# Autodesk Inventor assembly: forklift_1_0
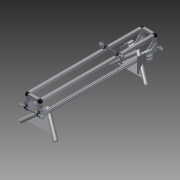
[picture p0: Inventor's stored thumbnail of the model, 180x180]
Saved by Autodesk Inventor 2011 (Build 150239000, 239)
## iProperties
Created: 2013-01-16
Part Number: forklift_1_0
Document SubType Name: Assembly
Designer: 917788
Author: 917788
## Documents named in this file (17)
- F:\Users\Christopher\Documents\GitHub\2013CAD\2013 robot\forklift\frame parts\forklift_1_0.iam
- F:\Users\Christopher\Documents\GitHub\2013CAD\2013 robot\forklift\frame parts\1tube_6.ipt
- F:\Users\Christopher\Documents\GitHub\2013CAD\2013 robot\forklift\frame parts\1tube_9.ipt
- F:\Users\Christopher\Documents\GitHub\2013CAD\2013 robot\forklift\frame parts\1tube_40.ipt
- F:\Users\Christopher\Documents\GitHub\2013CAD\2013 robot\forklift\frame parts\8020_40.ipt
- F:\Users\Christopher\Documents\GitHub\2013CAD\2013 robot\forklift\frame parts\8020_gussetplate.ipt
- F:\Users\Christopher\Documents\GitHub\2013CAD\2013 robot\forklift\Misc parts\3-way corner.ipt
- F:\Users\Christopher\Documents\GitHub\2013CAD\2013 robot\forklift\Misc parts\1.5_bolt_.25_20.ipt
- F:\Users\Christopher\Documents\GitHub\2013CAD\2013 robot\forklift\Misc parts\2_bolt_.25_20.ipt
- F:\Users\Christopher\Documents\GitHub\2013CAD\2013 robot\forklift\Misc parts\nut_.25_20.ipt
- F:\Users\Christopher\Documents\GitHub\2013CAD\2013 robot\forklift\frame parts\hook_right.iam
- F:\Users\Christopher\Documents\GitHub\2013CAD\2013 robot\forklift\frame parts\hook_left.iam
- F:\Users\Christopher\Documents\GitHub\2013CAD\2013 robot\forklift\Misc parts\.5inch_side_bearing.ipt
- F:\Users\Christopher\Documents\GitHub\2013CAD\2013 robot\forklift\frame parts\0.5unkeyedaxle_11.ipt
- F:\Users\Christopher\Documents\GitHub\2013CAD\2013 robot\forklift\Misc parts\.5_inch_axle_bushing.ipt
- F:\Users\Christopher\Documents\GitHub\2013CAD\2013 robot\forklift\frame parts\1.5inch_sprocket.ipt
- F:\Users\Christopher\Documents\GitHub\2013CAD\2013 robot\forklift\frame parts\corner_prop.ipt
## Components (137 placed, 16 different names)
1. 1tube_9:1 — Mate:9, Mate:10, Flush:8, Mate:11, Mate:12, Flush:9, Insert:3, Insert:4, Insert:44, Insert:51
2. 1tube_40:1 — Mate:7, Flush:7, Mate:8, Mate:20, Mate:21, Flush:18, Insert:2, Insert:12, Insert:43, Insert:136, Insert:137, Insert:144, Insert:145
3. 8020_40:1 — Flush:22, Flush:24, Mate:42, Flush:28, Mate:49, Flush:38, Flush:39, Mate:64, Mate:65
4. 8020_gussetplate:1 — Mate:50, Flush:40, Flush:41, Insert:84, Insert:85, Insert:86, Insert:87, Insert:88
5. 1tube_40:2 — Mate:13, Mate:14, Flush:10, Mate:22, Mate:23, Mate:24, Insert:6, Insert:8, Insert:52, Insert:58, Insert:138, Insert:139, Insert:146, Insert:147
6. 1tube_9:2 — Mate:25, Mate:26, Mate:27, Insert:9, Insert:10, Insert:67, Insert:71
7. 1tube_6:2 — Mate:1, Flush:4, Flush:5, Mate:46, Flush:36, Mate:48, Flush:37, Insert:1, Insert:42, Insert:77, Insert:104
8. 8020_40:2 — Mate:1, Flush:3, Flush:6, Flush:20, Flush:34, Mate:47, Flush:35, Flush:37, Mate:62, Mate:63
9. 8020_gussetplate:2 — Flush:24, Mate:43, Flush:31, Flush:32, Insert:53, Insert:54, Insert:55, Insert:56, Insert:57
10. 8020_gussetplate:3 — Mate:55, Flush:42, Flush:43, Insert:91, Insert:92, Insert:93, Insert:94, Insert:95
11. 8020_gussetplate:4 — Flush:5, Flush:6, Mate:46, Flush:36, Insert:89, Insert:90, Insert:96, Insert:97, Insert:98
12. 8020_gussetplate:5 — Flush:3, Flush:4, Mate:48, Insert:99, Insert:100, Insert:101, Insert:102, Insert:103
13. 8020_gussetplate:7 — Flush:22, Flush:29, Flush:30, Insert:32, Insert:33, Insert:34, Insert:35, Insert:36, Insert:158
14. 8020_gussetplate:8 — Mate:31, Flush:19, Flush:20, Insert:22, Insert:23, Insert:24, Insert:25, Insert:26
15. 8020_gussetplate:9 — Mate:37, Flush:25, Flush:26, Insert:60, Insert:61, Insert:62, Insert:63, Insert:64
16. 3-way corner:1 — Mate:11, Mate:12, Flush:9, Mate:13, Mate:14, Flush:10, Mate:52, Mate:53, Mate:54
17. 3-way corner:2 — Mate:7, Flush:7, Mate:8, Mate:9, Mate:10, Flush:8
18. 3-way corner:3 — Mate:20, Mate:21, Flush:18, Mate:25, Mate:28, Mate:29, Mate:30
19. 3-way corner:4 — Mate:22, Mate:23, Mate:24, Mate:26, Mate:27, Mate:44, Mate:51
20. 1tube_6:4 — Mate:28, Mate:29, Mate:30, Mate:31, Flush:19, Mate:37, Flush:25, Flush:26, Flush:34, Mate:47, Flush:35, Insert:11, Insert:68, Insert:111, Insert:112, Insert:119
21. 1tube_6:5 — Mate:42, Mate:43, Flush:28, Flush:29, Flush:30, Flush:31, Flush:32, Mate:44, Mate:51, Insert:7, Insert:59, Insert:113, Insert:114, Insert:120, Insert:158
22. 1tube_6:6 — Mate:49, Flush:38, Flush:39, Mate:50, Mate:52, Mate:53, Mate:54, Flush:40, Flush:41, Mate:55, Flush:42, Flush:43, Insert:5, Insert:50, Insert:73, Insert:105
23. 1.5_bolt_.25_20:1 — Insert:2
24. 1.5_bolt_.25_20:2 — Insert:1
25. 1.5_bolt_.25_20:3 — Insert:4
26. 1.5_bolt_.25_20:4 — Insert:3
27. 1.5_bolt_.25_20:5 — Insert:6
28. 1.5_bolt_.25_20:6 — Insert:11
29. 1.5_bolt_.25_20:7 — Insert:8
30. 1.5_bolt_.25_20:8 — Insert:9
31. 1.5_bolt_.25_20:9 — Insert:7
32. 1.5_bolt_.25_20:10 — Insert:10
33. 1.5_bolt_.25_20:13 — Insert:12
34. 1.5_bolt_.25_20:14 — Insert:5
35. 2_bolt_.25_20:8 — Insert:22
36. 2_bolt_.25_20:9 — Insert:23
37. 2_bolt_.25_20:10 — Insert:26
38. 2_bolt_.25_20:11 — Insert:24
39. 2_bolt_.25_20:12 — Insert:25
40. 2_bolt_.25_20:13 — Insert:35
41. 2_bolt_.25_20:14 — Insert:36
42. 2_bolt_.25_20:15 — Insert:34
43. 2_bolt_.25_20:16 — Insert:33
44. 2_bolt_.25_20:17 — Insert:32
45. nut_.25_20:4 — Insert:44
46. nut_.25_20:6 — Insert:50
47. nut_.25_20:7 — Insert:43
48. nut_.25_20:9 — Insert:52
49. nut_.25_20:10 — Insert:51
50. nut_.25_20:11 — Insert:53
51. nut_.25_20:17 — Insert:42
52. nut_.25_20:18 — Insert:63
53. nut_.25_20:19 — Insert:54
54. nut_.25_20:20 — Insert:61
55. nut_.25_20:21 — Insert:62
56. nut_.25_20:22 — Insert:57
57. nut_.25_20:23 — Insert:60
58. nut_.25_20:26 — Insert:59
59. nut_.25_20:27 — Insert:56
60. nut_.25_20:28 — Insert:64
61. nut_.25_20:30 — Insert:67
62. nut_.25_20:31 — Insert:55
63. nut_.25_20:33 — Insert:58
64. nut_.25_20:34 — Insert:71
65. nut_.25_20:35 — Insert:68
66. hook_right:1 [sub-assembly] — Flush:44, Flush:45, Mate:62, Mate:63
67. hook_left:1 [sub-assembly] — Flush:44, Mate:61, Mate:64, Mate:65
68. .5inch_side_bearing:3 — Insert:77, Insert:78, Insert:79, Insert:104, Insert:106, Insert:157
69. .5inch_side_bearing:4 — Insert:73, Insert:74, Insert:75, Insert:105, Insert:108
70. 1.5_bolt_.25_20:17 — Insert:78
71. 1.5_bolt_.25_20:18 — Insert:74
72. 1.5_bolt_.25_20:19 — Insert:75
73. 1.5_bolt_.25_20:20 — Insert:79
74. nut_.25_20:40 — Insert:95
75. 2_bolt_.25_20:18 — Insert:90
76. 2_bolt_.25_20:19 — Insert:84
77. 2_bolt_.25_20:20 — Insert:85
78. 2_bolt_.25_20:21 — Insert:86
79. 2_bolt_.25_20:22 — Insert:87
80. 2_bolt_.25_20:23 — Insert:96
81. 2_bolt_.25_20:24 — Insert:88
82. 2_bolt_.25_20:25 — Insert:89
83. 2_bolt_.25_20:28 — Insert:97
84. 2_bolt_.25_20:29 — Insert:98
85. nut_.25_20:41 — Insert:91
86. nut_.25_20:42 — Insert:92
87. nut_.25_20:43 — Insert:93
88. nut_.25_20:44 — Insert:101
89. nut_.25_20:45 — Insert:94
90. nut_.25_20:46 — Insert:102
91. nut_.25_20:47 — Insert:99
92. nut_.25_20:48 — Insert:103
93. nut_.25_20:49 — Insert:100
94. 0.5unkeyedaxle_11:1 — Insert:106, Insert:109, Insert:110
95. .5_inch_axle_bushing:1 — Insert:108
96. .5_inch_axle_bushing:2 — Insert:157
97. 1.5inch_sprocket:1 — Insert:109, Insert:122, Insert:124
98. 1.5inch_sprocket:2 — Insert:110, Insert:121, Insert:123
99. .5inch_side_bearing:5 — Insert:111, Insert:112, Insert:115, Insert:116, Insert:135
100. .5inch_side_bearing:6 — Insert:113, Insert:114, Insert:117, Insert:118, Insert:134
101. 1.5_bolt_.25_20:21 — Insert:115
102. 1.5_bolt_.25_20:22 — Insert:116
103. 1.5_bolt_.25_20:23 — Insert:117
104. 1.5_bolt_.25_20:24 — Insert:118
105. nut_.25_20:50 — Insert:119
106. nut_.25_20:51 — Insert:120
107. .5_inch_axle_bushing:3 — Insert:133
108. .5_inch_axle_bushing:4 — Insert:132
109. .5_inch_axle_bushing:5 — Insert:121
110. .5_inch_axle_bushing:6 — Insert:124
111. .5_inch_axle_bushing:7 — Insert:122
112. .5_inch_axle_bushing:8 — Insert:123
113. 1.5inch_sprocket:3 — Insert:128, Insert:131, Insert:132
114. 1.5inch_sprocket:4 — Insert:129, Insert:130, Insert:133
115. .5_inch_axle_bushing:9 — Insert:131
116. .5_inch_axle_bushing:10 — Insert:129, Insert:135
117. .5_inch_axle_bushing:11 — Insert:130
118. .5_inch_axle_bushing:12 — Insert:128, Insert:134
119. .5inch_side_bearing:7 — Insert:136, Insert:137, Insert:140, Insert:141, Insert:148
120. .5inch_side_bearing:8 — Insert:138, Insert:139, Insert:142, Insert:143
121. 1.5_bolt_.25_20:25 — Insert:140
122. 1.5_bolt_.25_20:26 — Insert:141
123. 1.5_bolt_.25_20:27 — Insert:142
124. 1.5_bolt_.25_20:28 — Insert:143
125. nut_.25_20:52 — Insert:146
126. nut_.25_20:53 — Insert:147
127. nut_.25_20:54 — Insert:145
128. nut_.25_20:55 — Insert:144
129. 0.5unkeyedaxle_11:2 — Insert:148, Insert:149, Insert:150, Insert:151
130. .5_inch_axle_bushing:13 — Insert:149
131. .5_inch_axle_bushing:14 — Insert:154
132. .5_inch_axle_bushing:15 — Insert:150, Insert:152
133. .5_inch_axle_bushing:17 — Insert:156
134. 1.5inch_sprocket:5 — Insert:151, Insert:156
135. 1.5inch_sprocket:6 — Insert:152, Insert:154
136. corner_prop:1 — Mate:61, Flush:45, Mate:66
137. corner_prop:2 — Mate:66
## Relationships (191: Insert 118, Mate 41, Flush 32)
- Mate:1: 1tube_6:2 ↔ 8020_40:2
- Flush:3: 8020_40:2 ↔ 8020_gussetplate:5
- Flush:4: 1tube_6:2 ↔ 8020_gussetplate:5
- Flush:5: 1tube_6:2 ↔ 8020_gussetplate:4
- Flush:6: 8020_40:2 ↔ 8020_gussetplate:4
- Mate:7: 1tube_40:1 ↔ 3-way corner:2
- Flush:7: 1tube_40:1 ↔ 3-way corner:2
- Mate:8: 1tube_40:1 ↔ 3-way corner:2
- Mate:9: 1tube_9:1 ↔ 3-way corner:2
- Mate:10: 1tube_9:1 ↔ 3-way corner:2
- Flush:8: 1tube_9:1 ↔ 3-way corner:2
- Mate:11: 1tube_9:1 ↔ 3-way corner:1
- Mate:12: 1tube_9:1 ↔ 3-way corner:1
- Flush:9: 1tube_9:1 ↔ 3-way corner:1
- Mate:13: 1tube_40:2 ↔ 3-way corner:1
- Mate:14: 1tube_40:2 ↔ 3-way corner:1
- Flush:10: 1tube_40:2 ↔ 3-way corner:1
- Mate:20: 1tube_40:1 ↔ 3-way corner:3
- Mate:21: 1tube_40:1 ↔ 3-way corner:3
- Flush:18: 1tube_40:1 ↔ 3-way corner:3
- Mate:22: 1tube_40:2 ↔ 3-way corner:4
- Mate:23: 1tube_40:2 ↔ 3-way corner:4
- Mate:24: 1tube_40:2 ↔ 3-way corner:4
- Mate:25: 1tube_9:2 ↔ 3-way corner:3
- Mate:26: 1tube_9:2 ↔ 3-way corner:4
- Mate:27: 1tube_9:2 ↔ 3-way corner:4
- Mate:28: 3-way corner:3 ↔ 1tube_6:4
- Mate:29: 3-way corner:3 ↔ 1tube_6:4
- Mate:30: 3-way corner:3 ↔ 1tube_6:4
- Mate:31: 8020_gussetplate:8 ↔ 1tube_6:4
- Flush:19: 8020_gussetplate:8 ↔ 1tube_6:4
- Flush:20: 8020_40:2 ↔ 8020_gussetplate:8
- Flush:22: 8020_40:1 ↔ 8020_gussetplate:7
- Flush:24: 8020_40:1 ↔ 8020_gussetplate:2
- Mate:37: 8020_gussetplate:9 ↔ 1tube_6:4
- Flush:25: 8020_gussetplate:9 ↔ 1tube_6:4
- Flush:26: 8020_gussetplate:9 ↔ 1tube_6:4
- Mate:42: 8020_40:1 ↔ 1tube_6:5
- Mate:43: 8020_gussetplate:2 ↔ 1tube_6:5
- Flush:28: 8020_40:1 ↔ 1tube_6:5
- Flush:29: 8020_gussetplate:7 ↔ 1tube_6:5
- Flush:30: 8020_gussetplate:7 ↔ 1tube_6:5
- Flush:31: 8020_gussetplate:2 ↔ 1tube_6:5
- Flush:32: 8020_gussetplate:2 ↔ 1tube_6:5
- Mate:44: 3-way corner:4 ↔ 1tube_6:5
- Flush:34: 8020_40:2 ↔ 1tube_6:4
- Mate:46: 1tube_6:2 ↔ 8020_gussetplate:4
- Mate:47: 8020_40:2 ↔ 1tube_6:4
- Flush:35: 8020_40:2 ↔ 1tube_6:4
- Flush:36: 1tube_6:2 ↔ 8020_gussetplate:4
- Mate:48: 1tube_6:2 ↔ 8020_gussetplate:5
- Flush:37: 1tube_6:2 ↔ 8020_40:2
- Mate:49: 8020_40:1 ↔ 1tube_6:6
- Flush:38: 8020_40:1 ↔ 1tube_6:6
- Flush:39: 8020_40:1 ↔ 1tube_6:6
- Mate:50: 8020_gussetplate:1 ↔ 1tube_6:6
- Mate:51: 3-way corner:4 ↔ 1tube_6:5
- Mate:52: 3-way corner:1 ↔ 1tube_6:6
- Mate:53: 3-way corner:1 ↔ 1tube_6:6
- Mate:54: 3-way corner:1 ↔ 1tube_6:6
- Flush:40: 8020_gussetplate:1 ↔ 1tube_6:6
- Flush:41: 8020_gussetplate:1 ↔ 1tube_6:6
- Mate:55: 8020_gussetplate:3 ↔ 1tube_6:6
- Flush:42: 8020_gussetplate:3 ↔ 1tube_6:6
- Flush:43: 8020_gussetplate:3 ↔ 1tube_6:6
- Insert:1: 1tube_6:2 ↔ 1.5_bolt_.25_20:2
- Insert:2: 1tube_40:1 ↔ 1.5_bolt_.25_20:1
- Insert:3: 1tube_9:1 ↔ 1.5_bolt_.25_20:4
- Insert:4: 1tube_9:1 ↔ 1.5_bolt_.25_20:3
- Insert:5: 1tube_6:6 ↔ 1.5_bolt_.25_20:14
- Insert:6: 1tube_40:2 ↔ 1.5_bolt_.25_20:5
- Insert:7: 1tube_6:5 ↔ 1.5_bolt_.25_20:9
- Insert:8: 1tube_40:2 ↔ 1.5_bolt_.25_20:7
- Insert:9: 1tube_9:2 ↔ 1.5_bolt_.25_20:8
- Insert:10: 1tube_9:2 ↔ 1.5_bolt_.25_20:10
- Insert:11: 1tube_6:4 ↔ 1.5_bolt_.25_20:6
- Insert:12: 1tube_40:1 ↔ 1.5_bolt_.25_20:13
- Insert:22: 8020_gussetplate:8 ↔ 2_bolt_.25_20:8
- Insert:23: 8020_gussetplate:8 ↔ 2_bolt_.25_20:9
- Insert:24: 8020_gussetplate:8 ↔ 2_bolt_.25_20:11
- Insert:25: 8020_gussetplate:8 ↔ 2_bolt_.25_20:12
- Insert:26: 8020_gussetplate:8 ↔ 2_bolt_.25_20:10
- Insert:32: 8020_gussetplate:7 ↔ 2_bolt_.25_20:17
- Insert:33: 8020_gussetplate:7 ↔ 2_bolt_.25_20:16
- Insert:34: 8020_gussetplate:7 ↔ 2_bolt_.25_20:15
- Insert:35: 8020_gussetplate:7 ↔ 2_bolt_.25_20:13
- Insert:36: 8020_gussetplate:7 ↔ 2_bolt_.25_20:14
- Insert:42: 1tube_6:2 ↔ nut_.25_20:17
- Insert:43: 1tube_40:1 ↔ nut_.25_20:7
- Insert:44: 1tube_9:1 ↔ nut_.25_20:4
- Insert:50: 1tube_6:6 ↔ nut_.25_20:6
- Insert:51: 1tube_9:1 ↔ nut_.25_20:10
- Insert:52: 1tube_40:2 ↔ nut_.25_20:9
- Insert:53: 8020_gussetplate:2 ↔ nut_.25_20:11
- Insert:54: 8020_gussetplate:2 ↔ nut_.25_20:19
- Insert:55: 8020_gussetplate:2 ↔ nut_.25_20:31
- Insert:56: 8020_gussetplate:2 ↔ nut_.25_20:27
- Insert:57: 8020_gussetplate:2 ↔ nut_.25_20:22
- Insert:58: 1tube_40:2 ↔ nut_.25_20:33
- Insert:59: 1tube_6:5 ↔ nut_.25_20:26
- Insert:60: 8020_gussetplate:9 ↔ nut_.25_20:23
- Insert:61: 8020_gussetplate:9 ↔ nut_.25_20:20
- Insert:62: 8020_gussetplate:9 ↔ nut_.25_20:21
- Insert:63: 8020_gussetplate:9 ↔ nut_.25_20:18
- Insert:64: 8020_gussetplate:9 ↔ nut_.25_20:28
- Insert:67: 1tube_9:2 ↔ nut_.25_20:30
- Insert:68: 1tube_6:4 ↔ nut_.25_20:35
- Insert:71: 1tube_9:2 ↔ nut_.25_20:34
- Insert:73: 1tube_6:6 ↔ .5inch_side_bearing:4
- Insert:74: .5inch_side_bearing:4 ↔ 1.5_bolt_.25_20:18
- Insert:75: .5inch_side_bearing:4 ↔ 1.5_bolt_.25_20:19
- Insert:77: 1tube_6:2 ↔ .5inch_side_bearing:3
- Insert:78: .5inch_side_bearing:3 ↔ 1.5_bolt_.25_20:17
- Insert:79: .5inch_side_bearing:3 ↔ 1.5_bolt_.25_20:20
- Insert:84: 8020_gussetplate:1 ↔ 2_bolt_.25_20:19
- Insert:85: 8020_gussetplate:1 ↔ 2_bolt_.25_20:20
- Insert:86: 8020_gussetplate:1 ↔ 2_bolt_.25_20:21
- Insert:87: 8020_gussetplate:1 ↔ 2_bolt_.25_20:22
- Insert:88: 8020_gussetplate:1 ↔ 2_bolt_.25_20:24
- Insert:89: 8020_gussetplate:4 ↔ 2_bolt_.25_20:25
- Insert:90: 8020_gussetplate:4 ↔ 2_bolt_.25_20:18
- Insert:91: 8020_gussetplate:3 ↔ nut_.25_20:41
- Insert:92: 8020_gussetplate:3 ↔ nut_.25_20:42
- Insert:93: 8020_gussetplate:3 ↔ nut_.25_20:43
- Insert:94: 8020_gussetplate:3 ↔ nut_.25_20:45
- Insert:95: 8020_gussetplate:3 ↔ nut_.25_20:40
- Insert:96: 8020_gussetplate:4 ↔ 2_bolt_.25_20:23
- Insert:97: 8020_gussetplate:4 ↔ 2_bolt_.25_20:28
- Insert:98: 8020_gussetplate:4 ↔ 2_bolt_.25_20:29
- Insert:99: 8020_gussetplate:5 ↔ nut_.25_20:47
- Insert:100: 8020_gussetplate:5 ↔ nut_.25_20:49
- Insert:101: 8020_gussetplate:5 ↔ nut_.25_20:44
- Insert:102: 8020_gussetplate:5 ↔ nut_.25_20:46
- Insert:103: 8020_gussetplate:5 ↔ nut_.25_20:48
- Insert:104: 1tube_6:2 ↔ .5inch_side_bearing:3
- Insert:105: 1tube_6:6 ↔ .5inch_side_bearing:4
- Insert:106 (-50.8 mm): .5inch_side_bearing:3 ↔ 0.5unkeyedaxle_11:1
- Insert:108: .5inch_side_bearing:4 ↔ .5_inch_axle_bushing:1
- Insert:109 (6.35 mm): 0.5unkeyedaxle_11:1 ↔ 1.5inch_sprocket:1
- Insert:110 (6.35 mm): 0.5unkeyedaxle_11:1 ↔ 1.5inch_sprocket:2
- Flush:44: hook_right:1 ↔ hook_left:1
- Insert:111: 1tube_6:4 ↔ .5inch_side_bearing:5
- Insert:112: 1tube_6:4 ↔ .5inch_side_bearing:5
- Insert:113: 1tube_6:5 ↔ .5inch_side_bearing:6
- Insert:114: 1tube_6:5 ↔ .5inch_side_bearing:6
- Insert:115: .5inch_side_bearing:5 ↔ 1.5_bolt_.25_20:21
- Insert:116: .5inch_side_bearing:5 ↔ 1.5_bolt_.25_20:22
- Insert:117: .5inch_side_bearing:6 ↔ 1.5_bolt_.25_20:23
- Insert:118: .5inch_side_bearing:6 ↔ 1.5_bolt_.25_20:24
- Insert:119: 1tube_6:4 ↔ nut_.25_20:50
- Insert:120: 1tube_6:5 ↔ nut_.25_20:51
- Insert:121: 1.5inch_sprocket:2 ↔ .5_inch_axle_bushing:5
- Insert:122: 1.5inch_sprocket:1 ↔ .5_inch_axle_bushing:7
- Insert:123: 1.5inch_sprocket:2 ↔ .5_inch_axle_bushing:8
- Insert:124: 1.5inch_sprocket:1 ↔ .5_inch_axle_bushing:6
- Insert:128 (-38.1 mm): 1.5inch_sprocket:3 ↔ .5_inch_axle_bushing:12
- Insert:129 (-38.1 mm): 1.5inch_sprocket:4 ↔ .5_inch_axle_bushing:10
- Insert:130: 1.5inch_sprocket:4 ↔ .5_inch_axle_bushing:11
- Insert:131: 1.5inch_sprocket:3 ↔ .5_inch_axle_bushing:9
- Insert:132: .5_inch_axle_bushing:4 ↔ 1.5inch_sprocket:3
- Insert:133: .5_inch_axle_bushing:3 ↔ 1.5inch_sprocket:4
- Insert:134: .5inch_side_bearing:6 ↔ .5_inch_axle_bushing:12
- Insert:135: .5inch_side_bearing:5 ↔ .5_inch_axle_bushing:10
- Insert:136: 1tube_40:1 ↔ .5inch_side_bearing:7
- Insert:137: 1tube_40:1 ↔ .5inch_side_bearing:7
- Insert:138: 1tube_40:2 ↔ .5inch_side_bearing:8
- Insert:139: 1tube_40:2 ↔ .5inch_side_bearing:8
- Insert:140: .5inch_side_bearing:7 ↔ 1.5_bolt_.25_20:25
- Insert:141: .5inch_side_bearing:7 ↔ 1.5_bolt_.25_20:26
- Insert:142: .5inch_side_bearing:8 ↔ 1.5_bolt_.25_20:27
- Insert:143: .5inch_side_bearing:8 ↔ 1.5_bolt_.25_20:28
- Insert:144: 1tube_40:1 ↔ nut_.25_20:55
- Insert:145: 1tube_40:1 ↔ nut_.25_20:54
- Insert:146: 1tube_40:2 ↔ nut_.25_20:52
- Insert:147: 1tube_40:2 ↔ nut_.25_20:53
- Insert:148 (-50.8 mm): .5inch_side_bearing:7 ↔ 0.5unkeyedaxle_11:2
- Insert:149: 0.5unkeyedaxle_11:2 ↔ .5_inch_axle_bushing:13
- Insert:150: 0.5unkeyedaxle_11:2 ↔ .5_inch_axle_bushing:15
- Insert:151 (6.35 mm): 0.5unkeyedaxle_11:2 ↔ 1.5inch_sprocket:5
- Insert:152 (6.35 mm): .5_inch_axle_bushing:15 ↔ 1.5inch_sprocket:6
- Insert:154: .5_inch_axle_bushing:14 ↔ 1.5inch_sprocket:6
- Insert:156: .5_inch_axle_bushing:17 ↔ 1.5inch_sprocket:5
- Mate:61: hook_left:1 ↔ corner_prop:1
- Flush:45 (12.7 mm): hook_right:1 ↔ corner_prop:1
- Mate:62: 8020_40:2 ↔ hook_right:1
- Mate:63: 8020_40:2 ↔ hook_right:1
- Mate:64: 8020_40:1 ↔ hook_left:1
- Mate:65: 8020_40:1 ↔ hook_left:1
- Insert:157: .5inch_side_bearing:3 ↔ .5_inch_axle_bushing:2
- Insert:158: 8020_gussetplate:7 ↔ 1tube_6:5
- Mate:66 (762 mm): corner_prop:1 ↔ corner_prop:2
